# Autodesk Inventor assembly: montagem_planta
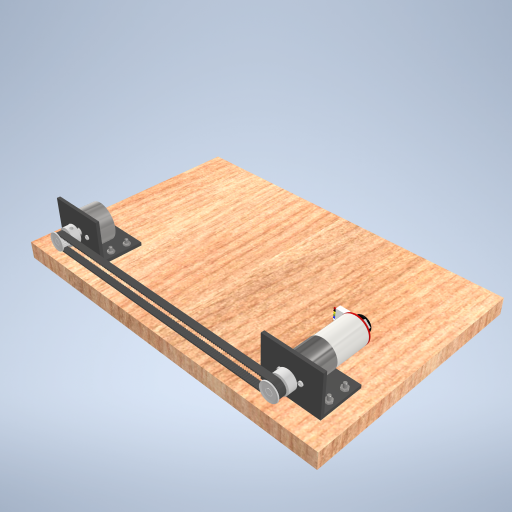
[picture p0: Inventor's stored thumbnail of the model, 512x512]
Saved by Autodesk Inventor 2023 (Build 270158000, 158)
## iProperties
Created: 2022-10-11
Part Number: montagem_planta
Document SubType Name: Assembly
Designer: klebe
Author: klebe
## Documents named in this file (16)
- C:\Users\klebe\OneDrive\Documents\GitHub\Eng_Meca\6º período\Lab_Analise\esteira\montagem_planta.iam
- C:\Users\klebe\OneDrive\Documents\GitHub\Eng_Meca\6º período\Lab_Analise\esteira\Base\base1.ipt
- C:\Users\klebe\OneDrive\Documents\GitHub\Eng_Meca\6º período\Lab_Analise\esteira\motor\JGA25-371_12VDC_85RPM.ipt
- C:\Users\klebe\OneDrive\Documents\GitHub\Eng_Meca\6º período\Lab_Analise\esteira\suporte\suporte.ipt
- C:\Users\klebe\OneDrive\Documents\GitHub\Eng_Meca\6º período\Lab_Analise\esteira\polia\poliaGT2 20B5.ipt
- C:\Users\klebe\OneDrive\Documents\GitHub\Eng_Meca\6º período\Lab_Analise\esteira\Acoplador\acoplador.ipt
- C:\Users\klebe\OneDrive\Documents\GitHub\Eng_Meca\6º período\Lab_Analise\esteira\Acoplador\suporte 2.ipt
- C:\Users\klebe\OneDrive\Documents\GitHub\Eng_Meca\6º período\Lab_Analise\esteira\motor\motor_sensor.ipt
- C:\Users\klebe\OneDrive\Documents\GitHub\Eng_Meca\6º período\Lab_Analise\esteira\Acoplador\acoplador_sensor.ipt
- C:\Users\klebe\OneDrive\Documents\Inventor\Content Center Files\R2023\en-US\ISO 7089\ISO 7089 - 3 - 140 HV(1).ipt
- C:\Users\klebe\OneDrive\Documents\Inventor\Content Center Files\R2023\en-US\ISO 4762(2)\ISO 4762 - M3 x 20ISO.ipt
- C:\Users\klebe\OneDrive\Documents\Inventor\Content Center Files\R2023\en-US\AS 1112 (4)\AS 1112 - M3(2).ipt
- C:\Users\klebe\OneDrive\Documents\GitHub\Eng_Meca\6º período\Lab_Analise\esteira\esteira\esteira_correia.ipt
- C:\Users\klebe\OneDrive\Documents\Inventor\Content Center Files\R2023\en-US\ISO 4032(2)\ISO 4032 - M3 - ISO.ipt
- C:\Users\klebe\OneDrive\Documents\Inventor\Content Center Files\R2023\en-US\DIN 7985 (H)\DIN 7985 (H) - M2x5-H.ipt
- C:\Users\klebe\OneDrive\Documents\Inventor\Content Center Files\R2023\en-US\DIN 7985 (H)\DIN 7985 (H) - M2x14-H.ipt
## Components (38 placed, 15 different names)
1. base1:1 — Mate:4, Mate:5, Mate:6, Mate:7, Mate:8, Mate:9, Mate:10, Mate:11, Mate:12, Mate:13, Mate:14, Mate:16, Mate:18, Mate:20, Mate:22, Mate:23, Mate:24, Mate:25, Mate:26, Mate:27, Mate:28, Mate:29, Mate:30, Mate:32, Mate:34, Mate:36
2. esteira_correia:1 — Rotational:3
3. motor — Rigid:5, Rigid:8
4. suporte:1 — Rigid:8, Mate:4, Mate:15, Mate:17, Mate:19, Mate:21, Insert:11, Insert:12
5. acoplador:1 — Rigid:5, Rotational:1, Rotational:3
6. poliaGT2 20B5:1 — Rotational:1
7. motor_sensor:1 — Rigid:6, Flush:2, Rigid:7
8. suporte 2:1 — Rigid:6, Mate:5, Mate:31, Mate:33, Mate:35, Mate:37, Insert:9, Insert:10
9. acoplador_sensor:1 — Flush:2, Rotational:2, Rigid:7
10. poliaGT2 20B5:2 — Rotational:2
11. DIN 7985 (H) M2x14-H:2 — Insert:12
12. DIN 7985 (H) M2x14-H:1 — Insert:11
13. AS 1112 (4) - Metric M3:4 — Mate:20, Mate:21
14. AS 1112 (4) - Metric M3:3 — Mate:18, Mate:19
15. AS 1112 (4) - Metric M3:2 — Mate:16, Mate:17
16. ISO 4762 M3 x 20:4 — Insert:4
17. ISO 4762 M3 x 20:3 — Insert:3
18. ISO 4762 M3 x 20:2 — Insert:2
19. ISO 7089 3:4 — Mate:12, Mate:13, Insert:4
20. ISO 7089 3:3 — Mate:10, Mate:11, Insert:3
21. ISO 7089 3:2 — Mate:8, Mate:9, Insert:2
22. AS 1112 (4) - Metric M3:1 — Mate:14, Mate:15
23. ISO 4762 M3 x 20:1 — Insert:1
24. ISO 7089 3:1 — Mate:6, Mate:7, Insert:1
25. DIN 7985 (H) M2x5-H:1 — Insert:9
26. DIN 7985 (H) M2x5-H:2 — Insert:10
27. ISO 4032 M3:4 — Mate:36, Mate:37
28. ISO 4032 M3:3 — Mate:34, Mate:35
29. ISO 4032 M3:2 — Mate:32, Mate:33
30. ISO 4762 M3 x 20:8 — Insert:8
31. ISO 4762 M3 x 20:7 — Insert:7
32. ISO 4762 M3 x 20:6 — Insert:6
33. ISO 7089 3:8 — Mate:28, Mate:29, Insert:8
34. ISO 7089 3:7 — Mate:26, Mate:27, Insert:7
35. ISO 7089 3:6 — Mate:24, Mate:25, Insert:6
36. ISO 4032 M3:1 — Mate:30, Mate:31
37. ISO 4762 M3 x 20:5 — Insert:5
38. ISO 7089 3:5 — Mate:22, Mate:23, Insert:5
## Relationships (54: Mate 34, Insert 12, WeldJoint 4, RevoluteJoint 3, Flush 1)
- Rigid:5 [WeldJoint]: motor ↔ acoplador:1
- Rotational:1 [RevoluteJoint]: acoplador:1 ↔ poliaGT2 20B5:1
- Rigid:6 [WeldJoint]: motor_sensor:1 ↔ suporte 2:1
- Flush:2: motor_sensor:1 ↔ acoplador_sensor:1
- Rotational:2 [RevoluteJoint]: acoplador_sensor:1 ↔ poliaGT2 20B5:2
- Rigid:7 [WeldJoint]: motor_sensor:1 ↔ acoplador_sensor:1
- Rigid:8 [WeldJoint]: motor ↔ suporte:1
- Mate:4: base1:1 ↔ suporte:1
- Mate:5: base1:1 ↔ suporte 2:1
- Mate:6: base1:1 ↔ ISO 7089 3:1
- Mate:7: base1:1 ↔ ISO 7089 3:1
- Mate:8: base1:1 ↔ ISO 7089 3:2
- Mate:9: base1:1 ↔ ISO 7089 3:2
- Mate:10: base1:1 ↔ ISO 7089 3:3
- Mate:11: base1:1 ↔ ISO 7089 3:3
- Mate:12: base1:1 ↔ ISO 7089 3:4
- Mate:13: base1:1 ↔ ISO 7089 3:4
- Insert:1: ISO 4762 M3 x 20:1 ↔ ISO 7089 3:1
- Insert:2: ISO 4762 M3 x 20:2 ↔ ISO 7089 3:2
- Insert:3: ISO 4762 M3 x 20:3 ↔ ISO 7089 3:3
- Insert:4: ISO 4762 M3 x 20:4 ↔ ISO 7089 3:4
- Mate:14: base1:1 ↔ AS 1112 (4) - Metric M3:1
- Mate:15: suporte:1 ↔ AS 1112 (4) - Metric M3:1
- Mate:16: base1:1 ↔ AS 1112 (4) - Metric M3:2
- Mate:17: suporte:1 ↔ AS 1112 (4) - Metric M3:2
- Mate:18: base1:1 ↔ AS 1112 (4) - Metric M3:3
- Mate:19: suporte:1 ↔ AS 1112 (4) - Metric M3:3
- Mate:20: base1:1 ↔ AS 1112 (4) - Metric M3:4
- Mate:21: suporte:1 ↔ AS 1112 (4) - Metric M3:4
- Rotational:3 [RevoluteJoint] (-1.5 mm): esteira_correia:1 ↔ acoplador:1
- Mate:22: base1:1 ↔ ISO 7089 3:5
- Mate:23: base1:1 ↔ ISO 7089 3:5
- Mate:24: base1:1 ↔ ISO 7089 3:6
- Mate:25: base1:1 ↔ ISO 7089 3:6
- Mate:26: base1:1 ↔ ISO 7089 3:7
- Mate:27: base1:1 ↔ ISO 7089 3:7
- Mate:28: base1:1 ↔ ISO 7089 3:8
- Mate:29: base1:1 ↔ ISO 7089 3:8
- Insert:5: ISO 4762 M3 x 20:5 ↔ ISO 7089 3:5
- Insert:6: ISO 4762 M3 x 20:6 ↔ ISO 7089 3:6
- Insert:7: ISO 4762 M3 x 20:7 ↔ ISO 7089 3:7
- Insert:8: ISO 4762 M3 x 20:8 ↔ ISO 7089 3:8
- Mate:30: base1:1 ↔ ISO 4032 M3:1
- Mate:31: suporte 2:1 ↔ ISO 4032 M3:1
- Mate:32: base1:1 ↔ ISO 4032 M3:2
- Mate:33: suporte 2:1 ↔ ISO 4032 M3:2
- Mate:34: base1:1 ↔ ISO 4032 M3:3
- Mate:35: suporte 2:1 ↔ ISO 4032 M3:3
- Mate:36: base1:1 ↔ ISO 4032 M3:4
- Mate:37: suporte 2:1 ↔ ISO 4032 M3:4
- Insert:9: suporte 2:1 ↔ DIN 7985 (H) M2x5-H:1
- Insert:10: suporte 2:1 ↔ DIN 7985 (H) M2x5-H:2
- Insert:11: suporte:1 ↔ DIN 7985 (H) M2x14-H:1
- Insert:12: suporte:1 ↔ DIN 7985 (H) M2x14-H:2
